# Autodesk Inventor assembly: gearbox_secondary_gear_as
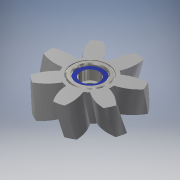
[picture p0: Inventor's stored thumbnail of the model, 180x180]
Saved by Autodesk Inventor 2019 (Build 230136000, 136)
## iProperties
Created: 2019-12-22
Part Number: gearbox_secondary_gear_as
Material: Типовые
Document SubType Name: Assembly
Designer: Петров Иван
Author: Петров Иван
## Documents named in this file (3)
- E:\IVAN\Ivan_desktop\Kvantorium\ROBOTS\Arm_manip\hardware\gearbox_secondary_gear_as.iam
- E:\IVAN\Ivan_desktop\Kvantorium\ROBOTS\Arm_manip\hardware\gearbox_secondary_gear.ipt
- E:\IVAN\Ivan_desktop\Kvantorium\ROBOTS\Arm_manip\hardware\Standart_things\Подшипник 4x8x3.ipt
## Components (2 placed, 2 different names)
1. Цилиндрическое зубчатое зацепление1:1 — Совмещение:1, Совмещение:2
2. Подшипник 4x8x3:1 — Совмещение:1, Совмещение:2
## Relationships (2: Mate 2)
- Совмещение:1 [Mate]: Цилиндрическое зубчатое зацепление1:1 ↔ Подшипник 4x8x3:1
- Совмещение:2 [Mate]: Цилиндрическое зубчатое зацепление1:1 ↔ Подшипник 4x8x3:1
